# Autodesk Inventor assembly: Assembly2
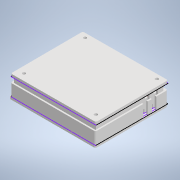
[picture p0: Inventor's stored thumbnail of the model, 180x180]
Saved by Autodesk Inventor 2020.2 (Build 242310000, 310)
## iProperties
Created: 2019-12-08
Part Number: Assembly2
Document SubType Name: Assembly
Designer: athiy
Author: athiy
## Documents named in this file (7)
- C:\Users\athiy\OneDrive\S2\01 KULIAH\SURG0094 Group Research Project\3D drawing\Assembly2.iam
- C:\Users\athiy\OneDrive\S2\01 KULIAH\SURG0094 Group Research Project\3D drawing\Part1.ipt
- C:\Users\athiy\OneDrive\S2\01 KULIAH\SURG0094 Group Research Project\3D drawing\Voice Recognition Module.ipt
- C:\Users\athiy\OneDrive\S2\01 KULIAH\SURG0094 Group Research Project\3D drawing\WICED Feather v12 v1\WICED Feather v12.iam
- C:\Users\athiy\OneDrive\S2\01 KULIAH\SURG0094 Group Research Project\3D drawing\Pin Headers\Pin Header 1x16 TH Pitch 2.54mm.ipt
- C:\Users\athiy\OneDrive\S2\01 KULIAH\SURG0094 Group Research Project\3D drawing\Pin Headers\Pin Header 1x12 TH Pitch 2.54mm.ipt
- C:\Users\athiy\OneDrive\S2\01 KULIAH\SURG0094 Group Research Project\3D drawing\Part2.ipt
## Components (6 placed, 6 different names)
1. Part1:1 — Mate:4, Mate:5, Mate:6, Mate:7
2. Voice Recognition Module:1 — Mate:4, Mate:5
3. WICED Feather v12:1 [sub-assembly] — Mate:6, Mate:7, Mate:8
4. Pin Header 1x16 TH Pitch 2.54mm:1
5. Pin Header 1x12 TH Pitch 2.54mm:1 — Mate:8
6. Part2:1
## Relationships (5: Mate 5)
- Mate:4: Part1:1 ↔ Voice Recognition Module:1
- Mate:5: Part1:1 ↔ Voice Recognition Module:1
- Mate:6: Part1:1 ↔ WICED Feather v12:1
- Mate:7: Part1:1 ↔ WICED Feather v12:1
- Mate:8: WICED Feather v12:1 ↔ Pin Header 1x12 TH Pitch 2.54mm:1
